# Autodesk Inventor assembly: Robot
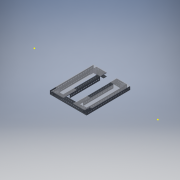
[picture p0: Inventor's stored thumbnail of the model, 180x180]
Saved by Autodesk Inventor 2016 (Build 200138000, 138)
## iProperties
Created: 2015-11-11
Part Number: Robot
Document SubType Name: Assembly
Designer: Julia
Author: Julia
## Documents named in this file (9)
- C:\Users\Aeolus\Documents\GitHub\RobotuxCAD\FTC CAD Parts\Robot Frame.iam
- C:\Users\Aeolus\Documents\GitHub\RobotuxCAD\FTC CAD Parts\Tetrix Parts\tetrix_739066_2012.ipt
- C:\Users\Aeolus\Documents\GitHub\RobotuxCAD\FTC CAD Parts\Tetrix Parts\tetrix_739068_2012.ipt
- C:\Users\Aeolus\Documents\GitHub\RobotuxCAD\FTC CAD Parts\Tetrix Parts\tetrix_739069_2012.ipt
- C:\Users\Aeolus\Documents\GitHub\RobotuxCAD\FTC CAD Parts\Tetrix Parts\tetrix_739281_corner_bra_2013.ipt
- C:\Users\Aeolus\Documents\GitHub\RobotuxCAD\FTC CAD Parts\Tetrix Parts\tetrix_739061_2012.ipt
- C:\Users\Aeolus\Documents\GitHub\RobotuxCAD\FTC CAD Parts\Lexan.ipt
- C:\Users\Aeolus\Documents\GitHub\RobotuxCAD\FTC CAD Parts\Tetrix Parts\tetrix_739387_2013.ipt
- C:\Users\Aeolus\Documents\GitHub\RobotuxCAD\FTC CAD Parts\Lexan_MIR.ipt
## Components (25 placed, 8 different names)
1. tetrix_739066_2012:1 — Mate:21, Mate:22, Mate:23, Mate:26, Mate:40, Mate:41, Mate:63, Mate:65, Mate:81, Mate:84, Mate:85
2. tetrix_739066_2012:2 — Mate:15, Mate:16, Mate:18, Mate:20, Mate:36, Mate:38, Mate:71, Mate:73, Mate:80, Mate:82, Mate:83, Flush:7
3. tetrix_739068_2012:2 — Mate:1, Mate:2, Mate:3, Mate:4, Mate:5, Mate:6, Mate:8, Mate:10, Mate:11, Mate:14, Mate:27, Mate:29, Mate:31, Mate:33, Mate:64, Mate:66, Mate:72, Mate:74, Mate:78, Mate:79, Mate:86, Mate:87, Mate:88, Mate:89, Flush:2
4. tetrix_739069_2012:1 — Mate:1, Mate:2, Mate:3, Mate:12, Mate:13, Mate:15, Mate:16, Mate:17, Mate:19, Mate:28, Mate:30, Mate:35, Mate:37, Flush:8
5. tetrix_739069_2012:2 — Mate:4, Mate:5, Mate:6, Mate:7, Mate:9, Mate:21, Mate:22, Mate:24, Mate:25, Mate:32, Mate:34, Mate:39, Mate:42, Flush:3
6. tetrix_739281_corner_bra_2013:1 — Mate:35, Mate:36, Mate:37, Mate:38
7. tetrix_739281_corner_bra_2013:2 — Mate:31, Mate:32, Mate:33, Mate:34
8. tetrix_739281_corner_bra_2013:3 — Mate:39, Mate:40, Mate:41, Mate:42
9. tetrix_739281_corner_bra_2013:4 — Mate:27, Mate:28, Mate:29, Mate:30
10. tetrix_739061_2012:3 — Mate:17, Mate:18, Mate:19, Mate:20
11. tetrix_739061_2012:4 — Mate:7, Mate:8, Mate:9, Mate:10
12. tetrix_739061_2012:5 — Mate:11, Mate:12, Mate:13, Mate:14
13. tetrix_739061_2012:6 — Mate:23, Mate:24, Mate:25, Mate:26
14. tetrix_739068_2012:5 — Flush:6
15. tetrix_739061_2012:11 — Mate:65
16. tetrix_739061_2012:12 — Mate:63, Mate:64, Mate:66, Mate:76, Mate:91
17. tetrix_739068_2012:6
18. tetrix_739061_2012:13 — Mate:71, Mate:73
19. tetrix_739061_2012:14 — Mate:72, Mate:74
20. Lexan:2 — Mate:76, Mate:90, Mate:91, Flush:2, Flush:3, Flush:6
21. tetrix_739387_2013:1 — Mate:80, Mate:82, Mate:83, Mate:92
22. tetrix_739387_2013:2 — Mate:78, Mate:88, Mate:89, Mate:90
23. tetrix_739387_2013:3 — Mate:81, Mate:84, Mate:85
24. tetrix_739387_2013:4 — Mate:79, Mate:86, Mate:87
25. Lexan_MIR:1 — Mate:92, Flush:7, Flush:8
## Relationships (79: Mate 74, Flush 5)
- Mate:1: tetrix_739068_2012:2 ↔ tetrix_739069_2012:1
- Mate:2: tetrix_739068_2012:2 ↔ tetrix_739069_2012:1
- Mate:3: tetrix_739068_2012:2 ↔ tetrix_739069_2012:1
- Mate:4: tetrix_739068_2012:2 ↔ tetrix_739069_2012:2
- Mate:5: tetrix_739068_2012:2 ↔ tetrix_739069_2012:2
- Mate:6: tetrix_739068_2012:2 ↔ tetrix_739069_2012:2
- Mate:7: tetrix_739069_2012:2 ↔ tetrix_739061_2012:4
- Mate:8: tetrix_739068_2012:2 ↔ tetrix_739061_2012:4
- Mate:9: tetrix_739069_2012:2 ↔ tetrix_739061_2012:4
- Mate:10: tetrix_739068_2012:2 ↔ tetrix_739061_2012:4
- Mate:11: tetrix_739068_2012:2 ↔ tetrix_739061_2012:5
- Mate:12: tetrix_739069_2012:1 ↔ tetrix_739061_2012:5
- Mate:13: tetrix_739069_2012:1 ↔ tetrix_739061_2012:5
- Mate:14: tetrix_739068_2012:2 ↔ tetrix_739061_2012:5
- Mate:15: tetrix_739066_2012:2 ↔ tetrix_739069_2012:1
- Mate:16: tetrix_739066_2012:2 ↔ tetrix_739069_2012:1
- Mate:17: tetrix_739069_2012:1 ↔ tetrix_739061_2012:3
- Mate:18: tetrix_739066_2012:2 ↔ tetrix_739061_2012:3
- Mate:19: tetrix_739069_2012:1 ↔ tetrix_739061_2012:3
- Mate:20: tetrix_739066_2012:2 ↔ tetrix_739061_2012:3
- Mate:21: tetrix_739066_2012:1 ↔ tetrix_739069_2012:2
- Mate:22: tetrix_739066_2012:1 ↔ tetrix_739069_2012:2
- Mate:23: tetrix_739066_2012:1 ↔ tetrix_739061_2012:6
- Mate:24: tetrix_739069_2012:2 ↔ tetrix_739061_2012:6
- Mate:25: tetrix_739069_2012:2 ↔ tetrix_739061_2012:6
- Mate:26: tetrix_739066_2012:1 ↔ tetrix_739061_2012:6
- Mate:27: tetrix_739068_2012:2 ↔ tetrix_739281_corner_bra_2013:4
- Mate:28: tetrix_739069_2012:1 ↔ tetrix_739281_corner_bra_2013:4
- Mate:29: tetrix_739068_2012:2 ↔ tetrix_739281_corner_bra_2013:4
- Mate:30: tetrix_739069_2012:1 ↔ tetrix_739281_corner_bra_2013:4
- Mate:31: tetrix_739068_2012:2 ↔ tetrix_739281_corner_bra_2013:2
- Mate:32: tetrix_739069_2012:2 ↔ tetrix_739281_corner_bra_2013:2
- Mate:33: tetrix_739068_2012:2 ↔ tetrix_739281_corner_bra_2013:2
- Mate:34: tetrix_739069_2012:2 ↔ tetrix_739281_corner_bra_2013:2
- Mate:35: tetrix_739069_2012:1 ↔ tetrix_739281_corner_bra_2013:1
- Mate:36: tetrix_739066_2012:2 ↔ tetrix_739281_corner_bra_2013:1
- Mate:37: tetrix_739069_2012:1 ↔ tetrix_739281_corner_bra_2013:1
- Mate:38: tetrix_739066_2012:2 ↔ tetrix_739281_corner_bra_2013:1
- Mate:39: tetrix_739069_2012:2 ↔ tetrix_739281_corner_bra_2013:3
- Mate:40: tetrix_739066_2012:1 ↔ tetrix_739281_corner_bra_2013:3
- Mate:41: tetrix_739066_2012:1 ↔ tetrix_739281_corner_bra_2013:3
- Mate:42: tetrix_739069_2012:2 ↔ tetrix_739281_corner_bra_2013:3
- [Mate]: tetrix_739068_2012:5 ↔ tetrix_739061_2012:11
- [Mate]: tetrix_739068_2012:5 ↔ tetrix_739061_2012:12
- [Mate]: tetrix_739068_2012:5 ↔ tetrix_739061_2012:11
- [Mate]: tetrix_739068_2012:5 ↔ tetrix_739061_2012:12
- Mate:63: tetrix_739066_2012:1 ↔ tetrix_739061_2012:12
- Mate:64: tetrix_739068_2012:2 ↔ tetrix_739061_2012:12
- Mate:65: tetrix_739066_2012:1 ↔ tetrix_739061_2012:11
- Mate:66: tetrix_739068_2012:2 ↔ tetrix_739061_2012:12
- [Mate]: tetrix_739068_2012:6 ↔ tetrix_739061_2012:13
- [Mate]: tetrix_739068_2012:6 ↔ tetrix_739061_2012:14
- [Mate]: tetrix_739068_2012:6 ↔ tetrix_739061_2012:13
- [Mate]: tetrix_739068_2012:6 ↔ tetrix_739061_2012:14
- Mate:71: tetrix_739066_2012:2 ↔ tetrix_739061_2012:13
- Mate:72: tetrix_739068_2012:2 ↔ tetrix_739061_2012:14
- Mate:73: tetrix_739066_2012:2 ↔ tetrix_739061_2012:13
- Mate:74: tetrix_739068_2012:2 ↔ tetrix_739061_2012:14
- Mate:76: tetrix_739061_2012:12 ↔ Lexan:2
- Mate:78: tetrix_739068_2012:2 ↔ tetrix_739387_2013:2
- Mate:79: tetrix_739068_2012:2 ↔ tetrix_739387_2013:4
- Mate:80: tetrix_739066_2012:2 ↔ tetrix_739387_2013:1
- Mate:81: tetrix_739066_2012:1 ↔ tetrix_739387_2013:3
- Mate:82: tetrix_739066_2012:2 ↔ tetrix_739387_2013:1
- Mate:83: tetrix_739066_2012:2 ↔ tetrix_739387_2013:1
- Mate:84: tetrix_739066_2012:1 ↔ tetrix_739387_2013:3
- Mate:85: tetrix_739066_2012:1 ↔ tetrix_739387_2013:3
- Mate:86: tetrix_739068_2012:2 ↔ tetrix_739387_2013:4
- Mate:87: tetrix_739068_2012:2 ↔ tetrix_739387_2013:4
- Mate:88: tetrix_739068_2012:2 ↔ tetrix_739387_2013:2
- Mate:89: tetrix_739068_2012:2 ↔ tetrix_739387_2013:2
- Mate:90: Lexan:2 ↔ tetrix_739387_2013:2
- Mate:91: tetrix_739061_2012:12 ↔ Lexan:2
- Flush:2: tetrix_739068_2012:2 ↔ Lexan:2
- Flush:3: tetrix_739069_2012:2 ↔ Lexan:2
- Flush:6: tetrix_739068_2012:5 ↔ Lexan:2
- Mate:92: tetrix_739387_2013:1 ↔ Lexan_MIR:1
- Flush:7: tetrix_739066_2012:2 ↔ Lexan_MIR:1
- Flush:8: tetrix_739069_2012:1 ↔ Lexan_MIR:1
## Named parameters: d110_d98_d97 = 0 mm, d111_d99_d94 = 0 mm, d112_d100_d95 = 0 mm, d113_d101_d96 = 0 mm, d118_d110_d98_d97 = 0 mm, d119_d111_d99_d94 = 0 mm, d120_d112_d100_d95 = 0 mm, d121_d113_d101_d96 = 0 mm
